# Autodesk Inventor assembly: stoł_2
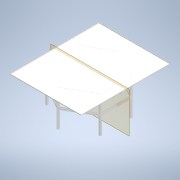
[picture p0: Inventor's stored thumbnail of the model, 180x180]
Saved by Autodesk Inventor 2021 (Build 250183000, 183)
## iProperties
Created: 2022-03-11
Part Number: stoł_2
Document SubType Name: Assembly
Designer: Norbert_Prokopiuk
_SolveAssemblyDoc: Frame Generator Solve Assembly
_Version: 25.0.0
Author: Norbert_Prokopiuk
## Documents named in this file (4)
- D:\studia\Magisterskie\pracownia robotyki\projekt\stoł_2.iam
- D:\studia\Magisterskie\pracownia robotyki\projekt\Part3.ipt
- D:\studia\Magisterskie\pracownia robotyki\projekt\stoł_2\Frame\Frame 1647020232368.iam
- D:\studia\Magisterskie\pracownia robotyki\projekt\stol_1.ipt
## Components (3 placed, 3 different names)
1. Part3:1
2. Frame 1647020232368:1 [sub-assembly] — Flush:1, Mate:2
3. stol_1:1 — Flush:1, Mate:1, Mate:2
## Relationships (3: Mate 2, Flush 1)
- Flush:1 (200 mm): Frame 1647020232368:1 ↔ stol_1:1
- Mate:1 (-1000 mm): stol_1:1
- Mate:2: Frame 1647020232368:1 ↔ stol_1:1
